# Autodesk Inventor assembly: frame
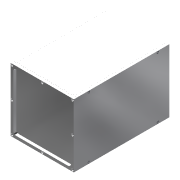
[picture p0: Inventor's stored thumbnail of the model, 180x180]
Saved by Autodesk Inventor 2018 (Build 220112000, 112)
## iProperties
Created: 2015-10-13
Part Number: frame
Document SubType Name: Assembly
Designer: Sawaiz
Author: Sawaiz
## Documents named in this file (9)
- C:\Users\sawaiz\OneDrive\projects\modularRICH\frame\frame.iam
- C:\Users\sawaiz\OneDrive\projects\modularRICH\frame\leftSide.ipt
- C:\Users\sawaiz\OneDrive\projects\modularRICH\frame\rightSide.ipt
- C:\Users\sawaiz\OneDrive\projects\modularRICH\frame\bottom.ipt
- C:\Users\sawaiz\OneDrive\projects\modularRICH\frame\front.ipt
- C:\Users\sawaiz\OneDrive\projects\modularRICH\frame\top.ipt
- C:\Users\sawaiz\OneDrive\projects\modularRICH\hardware\4-40x0.5in-flat.ipt
- C:\Users\sawaiz\OneDrive\projects\modularRICH\frame\frontClamp.ipt
- C:\Users\sawaiz\OneDrive\projects\modularRICH\modularRICH.xlsx
## Components (22 placed, 7 different names)
1. leftSide:1 — Flush:1, Symmetry:2, Flush:4, Flush:5, Mate:5, Mate:6, Mate:7, Mate:8, Symmetry:5, Flush:16, Mate:16
2. rightSide:1 — Flush:1, Symmetry:2, Flush:4, Mate:1, Mate:2, Mate:3, Mate:4, Symmetry:5, Angle:1, Flush:15, Mate:14, Flush:19, Mate:18
3. bottom:1 — Flush:2, Symmetry:1, Flush:3, Symmetry:4, Symmetry:6, Angle:2, Mate:13, Mate:17
4. front:1 — Mate:9, Mate:10, Mate:11, Mate:12, Angle:1, Angle:2, Mate:13, Flush:17, Mate:15, Flush:20, Flush:21, Flush:22, Flush:23
5. top:1 — Flush:2, Symmetry:1, Flush:3, Flush:5, Symmetry:4, Symmetry:6, Flush:15, Mate:14, Flush:18, Mate:19
6. 4-40x0.5in-flat:1 — Mate:7, Flush:11, Symmetry:3
7. 4-40x0.5in-flat:2 — Mate:11, Flush:12, Symmetry:7, Symmetry:8
8. 4-40x0.5in-flat:3 — Mate:12, Flush:12, Flush:13, Symmetry:8
9. 4-40x0.5in-flat:4 — Mate:1, Flush:6, Flush:7, Symmetry:3
10. 4-40x0.5in-flat:5 — Mate:10, Flush:13, Flush:14
11. 4-40x0.5in-flat:6 — Mate:2, Flush:7, Flush:8
12. 4-40x0.5in-flat:7 — Mate:4, Flush:6
13. 4-40x0.5in-flat:8 — Mate:3, Flush:8
14. 4-40x0.5in-flat:9 — Mate:6, Flush:10, Flush:11
15. 4-40x0.5in-flat:10 — Mate:9, Flush:14, Symmetry:7, Flush:17
16. 4-40x0.5in-flat:11 — Mate:8, Flush:9
17. 4-40x0.5in-flat:12 — Mate:5, Flush:9, Flush:10, Flush:16
18. frontClamp:1 — Flush:18, Flush:19, Mate:15
19. 4-40x0.5in-flat:13 — Mate:17, Flush:23
20. 4-40x0.5in-flat:14 — Mate:18, Flush:22
21. 4-40x0.5in-flat:15 — Mate:19, Flush:21
22. 4-40x0.5in-flat:16 — Mate:16, Flush:20
## Relationships (52: Flush 23, Mate 19, Symmetry 8, Angle 2)
- Flush:1: leftSide:1 ↔ rightSide:1
- Flush:2: bottom:1 ↔ top:1
- Symmetry:1: bottom:1 ↔ top:1
- Symmetry:2: leftSide:1 ↔ rightSide:1
- Flush:3: bottom:1 ↔ top:1
- Flush:4: leftSide:1 ↔ rightSide:1
- Flush:5: leftSide:1 ↔ top:1
- Mate:1: rightSide:1 ↔ 4-40x0.5in-flat:4
- Mate:2: rightSide:1 ↔ 4-40x0.5in-flat:6
- Mate:3: rightSide:1 ↔ 4-40x0.5in-flat:8
- Mate:4: rightSide:1 ↔ 4-40x0.5in-flat:7
- Flush:6: 4-40x0.5in-flat:4 ↔ 4-40x0.5in-flat:7
- Flush:7: 4-40x0.5in-flat:4 ↔ 4-40x0.5in-flat:6
- Flush:8: 4-40x0.5in-flat:6 ↔ 4-40x0.5in-flat:8
- Mate:5: leftSide:1 ↔ 4-40x0.5in-flat:12
- Mate:6: leftSide:1 ↔ 4-40x0.5in-flat:9
- Mate:7: leftSide:1 ↔ 4-40x0.5in-flat:1
- Mate:8: leftSide:1 ↔ 4-40x0.5in-flat:11
- Flush:9: 4-40x0.5in-flat:11 ↔ 4-40x0.5in-flat:12
- Flush:10: 4-40x0.5in-flat:9 ↔ 4-40x0.5in-flat:12
- Flush:11: 4-40x0.5in-flat:1 ↔ 4-40x0.5in-flat:9
- Symmetry:3: 4-40x0.5in-flat:1 ↔ 4-40x0.5in-flat:4
- Symmetry:4: bottom:1 ↔ top:1
- Symmetry:5: leftSide:1 ↔ rightSide:1
- Symmetry:6: bottom:1 ↔ top:1
- Mate:9: front:1 ↔ 4-40x0.5in-flat:10
- Mate:10: front:1 ↔ 4-40x0.5in-flat:5
- Mate:11: front:1 ↔ 4-40x0.5in-flat:2
- Mate:12: front:1 ↔ 4-40x0.5in-flat:3
- Flush:12: 4-40x0.5in-flat:2 ↔ 4-40x0.5in-flat:3
- Flush:13: 4-40x0.5in-flat:3 ↔ 4-40x0.5in-flat:5
- Flush:14: 4-40x0.5in-flat:5 ↔ 4-40x0.5in-flat:10
- Angle:1 (0 deg): rightSide:1 ↔ front:1
- Angle:2 (0 deg): bottom:1 ↔ front:1
- Symmetry:7: 4-40x0.5in-flat:2 ↔ 4-40x0.5in-flat:10
- Symmetry:8: 4-40x0.5in-flat:2 ↔ 4-40x0.5in-flat:3
- Mate:13: bottom:1 ↔ front:1
- Flush:15: rightSide:1 ↔ top:1
- Mate:14: rightSide:1 ↔ top:1
- Flush:16: leftSide:1 ↔ 4-40x0.5in-flat:12
- Flush:17: front:1 ↔ 4-40x0.5in-flat:10
- Flush:18: top:1 ↔ frontClamp:1
- Flush:19: rightSide:1 ↔ frontClamp:1
- Mate:15: front:1 ↔ frontClamp:1
- Mate:16: leftSide:1 ↔ 4-40x0.5in-flat:16
- Flush:20: front:1 ↔ 4-40x0.5in-flat:16
- Mate:17: bottom:1 ↔ 4-40x0.5in-flat:13
- Mate:18: rightSide:1 ↔ 4-40x0.5in-flat:14
- Mate:19: top:1 ↔ 4-40x0.5in-flat:15
- Flush:21: front:1 ↔ 4-40x0.5in-flat:15
- Flush:22: front:1 ↔ 4-40x0.5in-flat:14
- Flush:23: front:1 ↔ 4-40x0.5in-flat:13
## Named parameters: caseThickness = 6.35 mm, alignmentGrooveDepth = 1.5875 mm, alignmentGrooveClearance = 0.1016 mm, aerogelThickness = 30 mm, aerogelWidth = 110 mm, aerogelHeight = 110 mm, aerogelHolderDepth = 49.022 mm, height = 127 mm, width = 127 mm, depth = 203.2 mm, mirrorAngle = 2.5 deg, mirrorThickness = 3.175 mm, fresnelThickness = 0.254 mm, grooveDensity = 125, focalLength = 152.4 mm, ior = 1.49, centerThickness = 1.27 mm, fresnelAngle = 90 deg, fresnelEffectiveDiameter = 152.4 mm, frontPanelThickness = 1.5875 mm, fresnelGrooveWidth = 1.778 mm
